# Autodesk Inventor assembly: R-wing
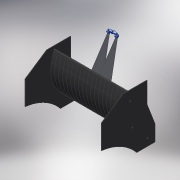
[picture p0: Inventor's stored thumbnail of the model, 180x180]
Saved by Autodesk Inventor 2018.2 (Build 222227000, 227)
## iProperties
Created: 2017-12-11
Part Number: R-wing
Material: 一般
Document SubType Name: Assembly
Designer: kuwano
Mass: 37579.8 g
Surface Area: 48667.5 cm^2
Volume: 32484 cm^3
Density: 1.15687 g/cm^3
Author: kuwano
## Documents named in this file (4)
- D:\kuwano\Documents\Inventor\KITformula\AeroCAD2018\CAD\Inventor\製作用CAD\R-wing\R-wing.iam
- D:\kuwano\Documents\Inventor\KITformula\AeroCAD2018\CAD\Inventor\製作用CAD\R-wing\parts\main_flap\main_flap.iam
- D:\kuwano\Documents\Inventor\KITformula\AeroCAD2018\CAD\Inventor\製作用CAD\R-wing\parts\end_plate.ipt
- D:\kuwano\Documents\Inventor\KITformula\AeroCAD2018\CAD\Inventor\製作用CAD\R-wing\parts\sub_flap\sub_flap.iam
## Components (4 placed, 3 different names)
1. main_flap:1 [sub-assembly] — メイト:1, メイト:2, メイト:3, メイト:4, メイト:5, メイト:7, メイト:8, メイト:9, メイト:10
2. sub_flap:1 [sub-assembly] — メイト:11, メイト:12
3. end_plate:1 — メイト:1, フラッシュ:1, フラッシュ:2, メイト:9, メイト:10
4. end_plate:2 — メイト:2, フラッシュ:1, フラッシュ:2, メイト:7, メイト:8, メイト:11, メイト:12
## Relationships (13: Mate 11, Flush 2)
- メイト:1 [Mate]: main_flap:1 ↔ end_plate:1
- メイト:2 [Mate]: main_flap:1 ↔ end_plate:2
- フラッシュ:1 [Flush]: end_plate:1 ↔ end_plate:2
- フラッシュ:2 [Flush]: end_plate:1 ↔ end_plate:2
- メイト:3 [Mate]: main_flap:1
- メイト:4 [Mate]: main_flap:1
- メイト:5 [Mate]: main_flap:1
- メイト:7 [Mate]: main_flap:1 ↔ end_plate:2
- メイト:8 [Mate]: main_flap:1 ↔ end_plate:2
- メイト:9 [Mate]: main_flap:1 ↔ end_plate:1
- メイト:10 [Mate]: main_flap:1 ↔ end_plate:1
- メイト:11 [Mate]: sub_flap:1 ↔ end_plate:2
- メイト:12 [Mate]: sub_flap:1 ↔ end_plate:2
